# Autodesk Inventor assembly: 組合2
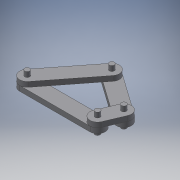
[picture p0: Inventor's stored thumbnail of the model, 180x180]
Saved by Autodesk Inventor 2019 (Build 230136000, 136)
## iProperties
Created: 2021-11-29
Part Number: 組合2
Material: 一般
Document SubType Name: Assembly
Designer: 10617
Author: 10617
## Documents named in this file (6)
- E:\cad2021\data\tmp\cad2021_hw\downloads\meARM\meARM_Inventor\組合2.iam
- E:\W11\Inventor\1.ipt
- E:\W11\Inventor\2.ipt
- E:\W11\Inventor\3.ipt
- E:\W11\Inventor\4.ipt
- E:\W11\Inventor\5.ipt
## Components (8 placed, 5 different names)
1. 1:1 — 貼合:1, 貼合:2, 貼合:3, 貼合:4, 貼合:10, 齊平:3, 貼合:11, 齊平:4
2. 2:1 — 貼合:3, 貼合:4, 貼合:5, 貼合:6
3. 3:1 — 貼合:5, 貼合:6, 貼合:7, 貼合:8, 齊平:1, 貼合:9, 齊平:2
4. 4:1 — 貼合:1, 貼合:2, 貼合:7
5. 5:1 — 貼合:8, 齊平:1
6. 5:2 — 貼合:9, 齊平:2
7. 5:3 — 貼合:11, 齊平:4
8. 5:4 — 貼合:10, 齊平:3
## Relationships (15: Mate 11, Flush 4)
- 貼合:1 [Mate]: 1:1 ↔ 4:1
- 貼合:2 [Mate]: 1:1 ↔ 4:1
- 貼合:3 [Mate]: 1:1 ↔ 2:1
- 貼合:4 [Mate]: 1:1 ↔ 2:1
- 貼合:5 [Mate]: 2:1 ↔ 3:1
- 貼合:6 [Mate]: 2:1 ↔ 3:1
- 貼合:7 [Mate]: 3:1 ↔ 4:1
- 貼合:8 [Mate]: 3:1 ↔ 5:1
- 齊平:1 [Flush] (-1 mm): 3:1 ↔ 5:1
- 貼合:9 [Mate]: 3:1 ↔ 5:2
- 齊平:2 [Flush] (-1 mm): 3:1 ↔ 5:2
- 貼合:10 [Mate]: 1:1 ↔ 5:4
- 齊平:3 [Flush] (-1 mm): 1:1 ↔ 5:4
- 貼合:11 [Mate]: 1:1 ↔ 5:3
- 齊平:4 [Flush] (-1 mm): 1:1 ↔ 5:3
